# Autodesk Inventor assembly: Robot Vacuum Final
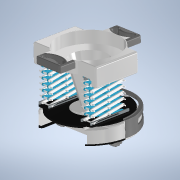
[picture p0: Inventor's stored thumbnail of the model, 180x180]
Saved by Autodesk Inventor 2021 (Build 250183000, 183)
## iProperties
Created: 2021-03-18
Part Number: Robot Vacuum Final
Document SubType Name: Assembly
Designer: Yuvraj Sandhu
Source: UnKnown
Author: Yuvraj Sandhu
## Documents named in this file (10)
- C:\Users\Darek\Desktop\Simulation Model\Robot Vacuum Final.iam
- C:\Users\Darek\Desktop\Simulation Model\Body.ipt
- C:\Users\Darek\Desktop\Simulation Model\Top plate 1.ipt
- C:\Users\Darek\Desktop\Simulation Model\Bumper.ipt
- C:\Users\Darek\Desktop\Simulation Model\Rear wheel.ipt
- C:\Users\Darek\Desktop\Simulation Model\Support axis.ipt
- C:\Users\Darek\Desktop\Simulation Model\Bottom plate.ipt
- C:\Users\Darek\Desktop\Simulation Model\Scissor Lift Prototype.iam
- C:\Users\Darek\Desktop\Simulation Model\Bin.ipt
- C:\Users\Darek\Desktop\Simulation Model\Sensor.ipt
## Components (15 placed, 10 different names)
1. Body — Mate:1, Mate:10, Mate:11, Mate:12, Mate:18, Mate:19, Mate:21, Mate:22, Mate:30, Mate:37, Mate:38, Mate:39, Mate:40
2. Top plate 1 — Mate:17, Flush:1, Flush:2, Mate:18, Mate:19, Mate:20, Flush:3, Flush:4, Mate:28, Mate:42, Flush:7
3. Bumper — Mate:12
4. Support axis 2
5. Rear wheel 2 — Mate:33, Mate:34
6. Bottom plate — Mate:1, Mate:10, Mate:11, Mate:31, Mate:32, Mate:33, Mate:34, Mate:35, Mate:36
7. Scissor Lift Prototype:1 [sub-assembly] — Mate:17, Flush:1, Flush:2, Flush:5, Mate:41, Flush:6
8. Scissor Lift Prototype:2 [sub-assembly] — Mate:20, Flush:3, Flush:4, Flush:5, Mate:27, Mate:29
9. Bin:1 — Mate:21, Mate:22, Mate:27, Mate:28, Mate:29, Mate:30
10. Rear wheel:3 — Mate:31, Mate:32
11. Rear wheel:4 — Mate:35, Mate:36
12. Sensor:4 — Mate:40, Mate:42, Flush:7
13. Sensor:5 — Mate:38, Mate:41, Flush:6, Mate:43, Angle:1, Flush:8
14. Sensor:6 — Mate:37, Flush:9, Flush:10
15. Sensor:7 — Mate:39, Mate:43, Angle:1, Flush:8, Flush:9, Flush:10
## Relationships (38: Mate 27, Flush 10, Angle 1)
- Mate:1: Body ↔ Bottom plate
- Mate:10: Body ↔ Bottom plate
- Mate:11: Body ↔ Bottom plate
- Mate:12: Body ↔ Bumper
- Mate:17: Top plate 1 ↔ Scissor Lift Prototype:1
- Flush:1: Top plate 1 ↔ Scissor Lift Prototype:1
- Flush:2: Top plate 1 ↔ Scissor Lift Prototype:1
- Mate:18: Body ↔ Top plate 1
- Mate:19: Body ↔ Top plate 1
- Mate:20: Top plate 1 ↔ Scissor Lift Prototype:2
- Flush:3: Top plate 1 ↔ Scissor Lift Prototype:2
- Flush:4: Top plate 1 ↔ Scissor Lift Prototype:2
- Mate:21: Body ↔ Bin:1
- Mate:22: Body ↔ Bin:1
- Flush:5: Scissor Lift Prototype:1 ↔ Scissor Lift Prototype:2
- Mate:27: Scissor Lift Prototype:2 ↔ Bin:1
- Mate:28: Top plate 1 ↔ Bin:1
- Mate:29: Scissor Lift Prototype:2 ↔ Bin:1
- Mate:30 (170.007 mm): Body ↔ Bin:1
- Mate:31: Bottom plate ↔ Rear wheel:3
- Mate:32 (20 mm): Bottom plate ↔ Rear wheel:3
- Mate:33: Rear wheel 2 ↔ Bottom plate
- Mate:34 (2.5 mm): Rear wheel 2 ↔ Bottom plate
- Mate:35: Bottom plate ↔ Rear wheel:4
- Mate:36 (5 mm): Bottom plate ↔ Rear wheel:4
- Mate:37: Body ↔ Sensor:6
- Mate:38: Body ↔ Sensor:5
- Mate:39: Body ↔ Sensor:7
- Mate:40: Body ↔ Sensor:4
- Mate:41 (30 mm): Scissor Lift Prototype:1 ↔ Sensor:5
- Flush:6: Scissor Lift Prototype:1 ↔ Sensor:5
- Mate:42 (30 mm): Top plate 1 ↔ Sensor:4
- Flush:7: Top plate 1 ↔ Sensor:4
- Mate:43 (40 mm): Sensor:5 ↔ Sensor:7
- Angle:1 (0 deg): Sensor:5 ↔ Sensor:7
- Flush:8 (100 mm): Sensor:5 ↔ Sensor:7
- Flush:9: Sensor:6 ↔ Sensor:7
- Flush:10 (-51 mm): Sensor:6 ↔ Sensor:7
